# Autodesk Inventor assembly: RSX Assembly
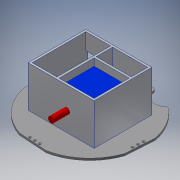
[picture p0: Inventor's stored thumbnail of the model, 180x180]
Saved by Autodesk Inventor 2016 (Build 200138000, 138)
## iProperties
Created: 2016-10-28
Part Number: RSX Assembly
Document SubType Name: Assembly
Designer: eschr_000
Author: eschr_000
## Documents named in this file (10)
- C:\Users\eschr_000\Documents\School\Hermes\CAD\RSX Assembly.iam
- C:\Users\eschr_000\Documents\School\Hermes\CAD\RSX Structure.ipt
- C:\Users\eschr_000\Documents\School\Hermes\CAD\VR Camera.ipt
- C:\Users\eschr_000\Documents\School\Hermes\CAD\Antenna.ipt
- C:\Users\eschr_000\Documents\School\Hermes\CAD\Pi Zero.iam
- C:\Users\eschr_000\Documents\School\Hermes\CAD\Hermes Cube.ipt
- C:\Users\eschr_000\Documents\School\Hermes\CAD\VR Camera Dome.ipt
- C:\Users\eschr_000\Documents\School\Hermes\CAD\Keep Out RSX Deck.ipt
- C:\Users\eschr_000\Documents\School\Hermes\CAD\RSX Deck.ipt
- C:\Users\eschr_000\Documents\School\Hermes\CAD\RSX Top.ipt
## Components (9 placed, 9 different names)
1. RSX Structure:1 — Mate:5, Mate:6, Mate:7, Mate:8, Mate:10, Flush:1, Mate:13, Mate:16, Mate:17, Mate:18, Symmetry:1, Mate:22, Mate:23, Mate:25, Mate:26, Mate:27, Mate:28, Mate:29, Mate:30, Mate:31, Mate:32
2. VR Camera:1 — Flush:1, Mate:13, Mate:14, Mate:15, Mate:25
3. Antenna:1 — Mate:6
4. Pi Zero:1 [sub-assembly] — Mate:5, Mate:7, Mate:8, Mate:32
5. Hermes Cube:1 — Mate:10, Symmetry:1, Mate:22, Mate:23
6. VR Camera Dome:1 — Mate:14, Mate:15
7. Keep Out RSX Deck:1 — Mate:16, Mate:17, Mate:18
8. RSX Top:1 — Mate:29, Mate:30, Mate:31
9. RSX Deck:1 — Mate:26, Mate:27, Mate:28
## Relationships (23: Mate 21, Flush 1, Symmetry 1)
- Mate:5: RSX Structure:1 ↔ Pi Zero:1
- Mate:6: RSX Structure:1 ↔ Antenna:1
- Mate:7: RSX Structure:1 ↔ Pi Zero:1
- Mate:8: RSX Structure:1 ↔ Pi Zero:1
- Mate:10: RSX Structure:1 ↔ Hermes Cube:1
- Flush:1: RSX Structure:1 ↔ VR Camera:1
- Mate:13 (28 mm): RSX Structure:1 ↔ VR Camera:1
- Mate:14: VR Camera:1 ↔ VR Camera Dome:1
- Mate:15: VR Camera:1 ↔ VR Camera Dome:1
- Mate:16: RSX Structure:1 ↔ Keep Out RSX Deck:1
- Mate:17: RSX Structure:1 ↔ Keep Out RSX Deck:1
- Mate:18: RSX Structure:1 ↔ Keep Out RSX Deck:1
- Symmetry:1: RSX Structure:1 ↔ Hermes Cube:1
- Mate:22: RSX Structure:1 ↔ Hermes Cube:1
- Mate:23: RSX Structure:1 ↔ Hermes Cube:1
- Mate:25 (38.1 mm): RSX Structure:1 ↔ VR Camera:1
- Mate:26: RSX Structure:1 ↔ RSX Deck:1
- Mate:27: RSX Structure:1 ↔ RSX Deck:1
- Mate:28: RSX Structure:1 ↔ RSX Deck:1
- Mate:29: RSX Structure:1 ↔ RSX Top:1
- Mate:30: RSX Structure:1 ↔ RSX Top:1
- Mate:31: RSX Structure:1 ↔ RSX Top:1
- Mate:32: RSX Structure:1 ↔ Pi Zero:1
